# Autodesk Inventor assembly: NewSmallSize(2xl)
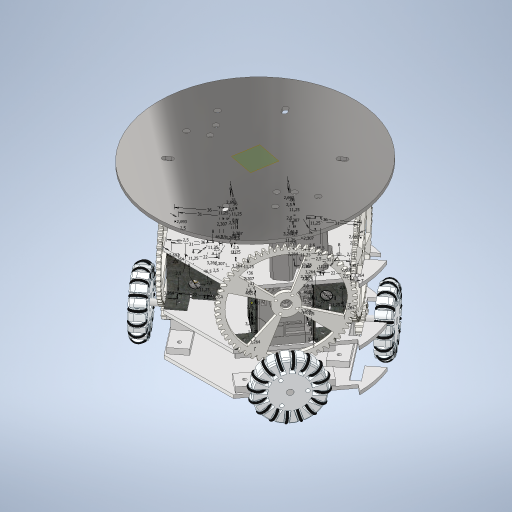
[picture p0: Inventor's stored thumbnail of the model, 512x512]
Saved by Autodesk Inventor 2023 (Build 270158000, 158)
## iProperties
Created: 2022-09-27
Part Number: NewSmallSize(2xl)
Document SubType Name: Assembly
Designer: hiago.sodre
Author: hiago.sodre
## Documents named in this file (6)
- C:\Users\hiago.sodre\Downloads\MODELO2XL-430\Model_2XL430-W250-T\NewSmallSize(2xl).iam
- C:\Users\hiago.sodre\Downloads\MODELO2XL-430\Model_2XL430-W250-T\soporte_eje_omni.ipt
- C:\Users\hiago.sodre\Downloads\MODELO2XL-430\Model_2XL430-W250-T\EjeRueda.iam
- C:\Users\hiago.sodre\Downloads\MODELO2XL-430\Model_2XL430-W250-T\2XL-430montado.iam
- C:\Users\hiago.sodre\Downloads\MODELO2XL-430\Model_2XL430-W250-T\newbaseeditado.ipt
- C:\Users\hiago.sodre\Downloads\MODELO2XL-430\Model_2XL430-W250-T\Toplayer.ipt
## Components (16 placed, 5 different names)
1. soporte_eje_omni:1 — De rotación:1, De rotación:5, Coincidencia:20
2. soporte_eje_omni:2 — Mate:8, De rotación:2, Rígido:1
3. EjeRueda:1 [sub-assembly] — Mate:8
4. EjeRueda:2 [sub-assembly] — De rotación:1
5. EjeRueda:3 [sub-assembly] — Mate:15
6. EjeRueda:4 [sub-assembly] — Mate:11
7. soporte_eje_omni:5 — Mate:11, De rotación:3
8. soporte_eje_omni:6 — Mate:15, De rotación:4
9. 2XL-430montado:1 [sub-assembly] — Coincidencia:16, Coincidencia:21, Coincidencia:23
10. 2XL-430montado:2 [sub-assembly] — Coincidencia:17, Coincidencia:22
11. 2XL-430montado:3 [sub-assembly] — Coincidencia:18, Coincidencia:24
12. 2XL-430montado:4 [sub-assembly] — Coincidencia:19, Coincidencia:25
13. newbaseeditado:2 — Rígido:1, Coincidencia:20
14. Toplayer:1
15. newbaseeditado:3 — Coincidencia:16, De rotación:2, Coincidencia:17, De rotación:3, Coincidencia:18, De rotación:4, Coincidencia:19, De rotación:5
16. newbaseeditado:4 — Coincidencia:21, Coincidencia:22, Coincidencia:23, Coincidencia:24, Coincidencia:25
## Relationships (19: Mate 13, RevoluteJoint 5, WeldJoint 1)
- Mate:8: soporte_eje_omni:2 ↔ EjeRueda:1
- Mate:11: EjeRueda:4 ↔ soporte_eje_omni:5
- Mate:15: EjeRueda:3 ↔ soporte_eje_omni:6
- De rotación:1 [RevoluteJoint]: soporte_eje_omni:1 ↔ EjeRueda:2
- Coincidencia:16 [Mate]: 2XL-430montado:1 ↔ newbaseeditado:3
- De rotación:2 [RevoluteJoint]: soporte_eje_omni:2 ↔ newbaseeditado:3
- Coincidencia:17 [Mate]: 2XL-430montado:2 ↔ newbaseeditado:3
- De rotación:3 [RevoluteJoint]: soporte_eje_omni:5 ↔ newbaseeditado:3
- Coincidencia:18 [Mate]: 2XL-430montado:3 ↔ newbaseeditado:3
- De rotación:4 [RevoluteJoint]: soporte_eje_omni:6 ↔ newbaseeditado:3
- Coincidencia:19 [Mate]: 2XL-430montado:4 ↔ newbaseeditado:3
- De rotación:5 [RevoluteJoint]: soporte_eje_omni:1 ↔ newbaseeditado:3
- Rígido:1 [WeldJoint]: soporte_eje_omni:2 ↔ newbaseeditado:2
- Coincidencia:20 [Mate]: soporte_eje_omni:1 ↔ newbaseeditado:2
- Coincidencia:21 [Mate]: 2XL-430montado:1 ↔ newbaseeditado:4
- Coincidencia:22 [Mate]: 2XL-430montado:2 ↔ newbaseeditado:4
- Coincidencia:23 [Mate]: 2XL-430montado:1 ↔ newbaseeditado:4
- Coincidencia:24 [Mate]: 2XL-430montado:3 ↔ newbaseeditado:4
- Coincidencia:25 [Mate]: 2XL-430montado:4 ↔ newbaseeditado:4
